# Autodesk Inventor assembly: Z-Axis Assembly
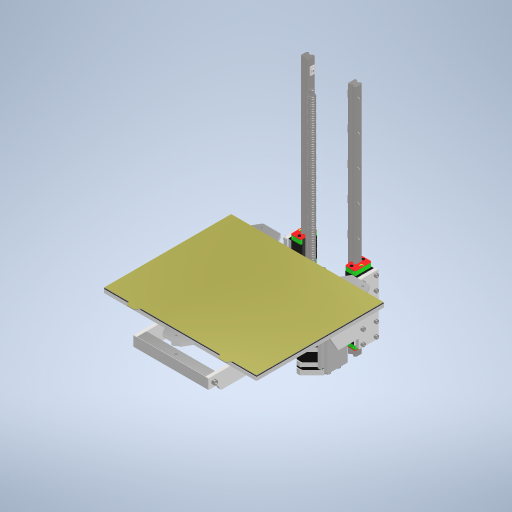
[picture p0: Inventor's stored thumbnail of the model, 512x512]
Saved by Autodesk Inventor 2024 (Build 280153000, 153)
## iProperties
Created: 2024-08-01
Part Number: Z-Axis Assembly
Document SubType Name: Assembly
Designer: Ishaan
Author: Ishaan
## Documents named in this file (32)
- E:\Projects\Axiom--IDEX-3D-Printer\CAD\03 - Z-Axis\Z-Axis Assembly.iam
- E:\Projects\Axiom--IDEX-3D-Printer\CAD\03 - Z-Axis\Z-Axis Motor Plate.ipt
- E:\Projects\Axiom--IDEX-3D-Printer\CAD\00 - COTS Components\FK10\FK10-C5\FK10-C5\FK10-C5.iam
- E:\Projects\Axiom--IDEX-3D-Printer\CAD\00 - COTS Components\5x8 Shaft Coupler\Flexible Coupling 5mm x 8mm.ipt
- E:\Projects\Axiom--IDEX-3D-Printer\CAD\00 - COTS Components\FK10\FK10-C5\Гайка М10х1\Гайка М10х1.iam
- E:\Projects\Axiom--IDEX-3D-Printer\CAD\00 - COTS Components\SFU1204 Ballscrew\1204 Ballscrew.ipt
- E:\Projects\Axiom--IDEX-3D-Printer\CAD\00 - COTS Components\NEMA 17 - Z-Axis Long\NEMA 17 Z-axis Long.ipt
- E:\Projects\Axiom--IDEX-3D-Printer\CAD\03 - Z-Axis\Z-Axis Motor Spacer.ipt
- E:\Projects\Axiom--IDEX-3D-Printer\CAD\00 - COTS Components\NEMA 17 - Z-Axis Short\NEMA 17 Z-axis Short.ipt
- E:\Projects\Axiom--IDEX-3D-Printer\CAD\00 - COTS Components\HGR15 Z-Axis Rail\HGR15-R-700mm\HGR15-R-700mm.iam
- E:\Projects\Axiom--IDEX-3D-Printer\CAD\03 - Z-Axis\Bed Heater.ipt
- E:\Projects\Axiom--IDEX-3D-Printer\CAD\03 - Z-Axis\Bed Magnet.ipt
- E:\Projects\Axiom--IDEX-3D-Printer\CAD\03 - Z-Axis\PEI Bed Surface.ipt
- E:\Projects\Axiom--IDEX-3D-Printer\CAD\03 - Z-Axis\Print Bed.ipt
- E:\Projects\Axiom--IDEX-3D-Printer\CAD\00 - COTS Components\HGH15CA Carriage Block\HGH15CA Hiwin Linear block by proma\HGH15CA Hiwin Linear block by proma.ipt
- E:\Projects\Axiom--IDEX-3D-Printer\CAD\03 - Z-Axis\Z-Axis Bed Plates.ipt
- E:\Projects\Axiom--IDEX-3D-Printer\CAD\00 - COTS Components\2020 Bed Front Extrusion\HFSC5-2020-138.ipt
- E:\Projects\Axiom--IDEX-3D-Printer\CAD\00 - COTS Components\2040 Bed Rear Extrusion\HFSF5-2040-138.ipt
- E:\Projects\Axiom--IDEX-3D-Printer\CAD\00 - COTS Components\1204 Ballscrew Nut\Ballscrew nut 1204 by proma\Ballscrew nut 1204 by proma.ipt
- E:\Projects\Axiom--IDEX-3D-Printer\CAD\03 - Z-Axis\Print Bed Washers.ipt
- E:\Projects\Axiom--IDEX-3D-Printer\CAD\03 - Z-Axis\Z-Axis Nut and Bed Plate RevII.ipt
- E:\Projects\Axiom--IDEX-3D-Printer\CAD\00 - COTS Components\Hardware\M4 T SLOT NUT.ipt
- E:\Projects\Axiom--IDEX-3D-Printer\CAD\00 - COTS Components\Hardware\SHCSM4x14.ipt
- E:\Projects\Axiom--IDEX-3D-Printer\CAD\00 - COTS Components\Hardware\SHCSM5x16.ipt
- E:\Projects\Axiom--IDEX-3D-Printer\CAD\00 - COTS Components\Hardware\SHCSM5x12.ipt
- E:\Projects\Axiom--IDEX-3D-Printer\CAD\00 - COTS Components\Hardware\SHCSM4x10.ipt
- E:\Projects\Axiom--IDEX-3D-Printer\CAD\00 - COTS Components\Hardware\M4 LOCKNUT.ipt
- E:\Projects\Axiom--IDEX-3D-Printer\CAD\00 - COTS Components\Hardware\SHCSM3x8.ipt
- E:\Projects\Axiom--IDEX-3D-Printer\CAD\00 - COTS Components\Hardware\Low Profile M5x12.ipt
- E:\Projects\Axiom--IDEX-3D-Printer\CAD\00 - COTS Components\2040 Z-motor Supports\HFSF5-2040-85.ipt
- E:\Projects\Axiom--IDEX-3D-Printer\CAD\02 - Frame\Printer Base Plate RevII.ipt
- E:\Projects\Axiom--IDEX-3D-Printer\CAD\00 - COTS Components\4080 Z-rail Extrusion\HFSP5-4080-475.ipt
## Components (123 placed, 31 different names)
1. Z-Axis Motor Plate:1 — Insert:1, Insert:2, Insert:7, Insert:8, Insert:74, Insert:75, Insert:76, Insert:77, Insert:86, Insert:87, Insert:88, Insert:89
2. FK10-C5:1 [sub-assembly] — Insert:1, Insert:2, Insert:3, Insert:5, Insert:78, Insert:79, Insert:80, Insert:81
3. Flexible Coupling 5mm x 8mm:1 — Insert:6
4. Гайка М10х1:1 [sub-assembly] — Insert:3
5. 1204 Ballscrew:1 — Insert:5, Insert:6, Z POSITION
6. NEMA 17 Z-axis Long:1 — Insert:9, Insert:10
7. Z-Axis Motor Spacer:1 — Insert:7, Insert:8, Insert:9, Insert:10, Insert:11, Insert:12, Insert:82, Angle:4, Insert:83, Angle:5, Insert:84, Angle:6, Insert:85, Angle:7, Insert:106, Insert:107, Insert:108, Insert:109
8. NEMA 17 Z-axis Short:1 — Insert:11, Insert:12
9. HFSF5-2040-85:1 — Insert:17
10. HFSF5-2040-85:2 — Insert:18
11. Printer Base Plate RevII:1 — Insert:17, Insert:18
12. HFSP5-4080-475:1
13. HGR15-R-700mm:1 [sub-assembly] — Flush:2, Flush:3, Mate:16, Mate:17, Mate:18, Mate:19
14. HGR15-R-700mm:2 [sub-assembly] — Flush:2, Flush:3, Mate:12, Mate:13, Mate:14, Mate:15, Insert:53
15. Bed Heater:1 — Mate:8, Flush:6, Flush:7
16. Bed Magnet:1 — Mate:4, Flush:4, Mate:5, Mate:6
17. PEI Bed Surface:1 — Mate:6, Flush:5, Flush:8, Flush:9
18. Print Bed:1 — Mate:4, Flush:4, Mate:5, Flush:5, Mate:8, Flush:6, Flush:7, Flush:8, Mate:20, Insert:49, Insert:50, Insert:51, Mate:23, Mate:24
19. HGH15CA Hiwin Linear block by proma:1 — Mate:16, Mate:17, Insert:33, Insert:34, Insert:35, Insert:36
20. HGH15CA Hiwin Linear block by proma:2 — Mate:14, Mate:15, Insert:21, Insert:22, Insert:23, Insert:24
21. HGH15CA Hiwin Linear block by proma:3 — Mate:18, Mate:19, Insert:29, Insert:30, Insert:31, Insert:32
22. HGH15CA Hiwin Linear block by proma:4 — Mate:12, Mate:13, Insert:25, Insert:26, Insert:27, Insert:28
23. Z-Axis Bed Plates:1 — Insert:21, Insert:22, Insert:23, Insert:24, Insert:25, Insert:26, Insert:27, Insert:28, Insert:37, Angle:1, Flush:9, Insert:39, Insert:40, Insert:60, Insert:61, Insert:62, Insert:90, Insert:91, Insert:92, Insert:93, Insert:94, Insert:95, Insert:96, Insert:97
24. Z-Axis Bed Plates:2 — Insert:29, Insert:30, Insert:31, Insert:32, Insert:33, Insert:34, Insert:35, Insert:36, Insert:38, Insert:41, Insert:42, Insert:63, Insert:64, Insert:65, Insert:98, Insert:99, Insert:100, Insert:101, Insert:102, Insert:103, Insert:104, Insert:105
25. HFSC5-2020-138:1 — Insert:37, Insert:38, Angle:1, Mate:20
26. HFSF5-2040-138:1 — Insert:39, Insert:40, Insert:41, Insert:42
27. Z-Axis Nut and Bed Plate RevII:1 — Mate:23, Mate:24, Insert:66, Insert:67, Insert:68, Insert:69, Insert:70, Insert:71, Insert:72, Insert:73
28. Ballscrew nut 1204 by proma:1 — Z POSITION, Insert:54, Insert:55, Insert:56, Insert:57, Insert:58, Insert:59
29. Print Bed Washers:1 — Insert:49
30. Print Bed Washers:2 — Insert:50
31. Print Bed Washers:3 — Insert:51
32. SHCSM4x10:13 — Insert:103
33. SHCSM4x10:14 — Insert:102
34. SHCSM4x10:15 — Insert:100
35. SHCSM4x10:16 — Insert:99
36. SHCSM4x10:17 — Insert:98
37. SHCSM4x10:18 — Insert:101
38. SHCSM4x10:19 — Insert:104
39. SHCSM4x10:20 — Insert:105
40. SHCSM3x8:1 — Insert:106
41. SHCSM3x8:2 — Insert:107
42. SHCSM3x8:3 — Insert:109
43. SHCSM3x8:4 — Insert:108
44. Low Profile M5x12:1
45. Low Profile M5x12:2
46. Low Profile M5x12:3
47. Low Profile M5x12:4
48. SHCSM5x12:1 — Insert:66
49. SHCSM5x12:2 — Insert:67
50. SHCSM5x12:3 — Insert:73
51. SHCSM5x12:4 — Insert:69
52. SHCSM5x12:5 — Insert:68
53. SHCSM5x12:6 — Insert:70
54. SHCSM5x12:7 — Insert:72
55. SHCSM5x12:8 — Insert:71
56. SHCSM5x16:7 — Insert:74
57. SHCSM5x16:8 — Insert:75
58. SHCSM5x16:9 — Insert:76
59. SHCSM5x16:10 — Insert:77
60. SHCSM4x10:1 — Insert:78
61. SHCSM4x10:2 — Insert:79
62. SHCSM4x10:3 — Insert:80
63. SHCSM4x10:4 — Insert:81
64. M4 LOCKNUT:1 — Insert:82, Angle:4
65. M4 LOCKNUT:2 — Insert:83, Angle:5
66. M4 LOCKNUT:3 — Insert:84, Angle:6
67. M4 LOCKNUT:4 — Insert:85, Angle:7
68. SHCSM4x14:23 — Insert:86
69. SHCSM4x14:24 — Insert:87
70. SHCSM4x14:25 — Insert:88
71. SHCSM4x14:26 — Insert:89
72. SHCSM4x10:5 — Insert:94
73. SHCSM4x10:6 — Insert:95
74. SHCSM4x10:7 — Insert:96
75. SHCSM4x10:8 — Insert:97
76. SHCSM4x10:9 — Insert:93
77. SHCSM4x10:10 — Insert:92
78. SHCSM4x10:11 — Insert:91
79. SHCSM4x10:12 — Insert:90
80. SHCSM5x16:1 — Insert:60
81. SHCSM5x16:2 — Insert:61
82. SHCSM5x16:3 — Insert:62
83. SHCSM5x16:4 — Insert:63
84. SHCSM5x16:5 — Insert:65
85. SHCSM5x16:6 — Insert:64
86. SHCSM4x14:17 — Insert:56
87. SHCSM4x14:18 — Insert:57
88. SHCSM4x14:19 — Insert:55
89. SHCSM4x14:20 — Insert:58
90. SHCSM4x14:21 — Insert:54
91. SHCSM4x14:22 — Insert:59
92. SHCSM4x14:1 — Insert:53, Mate:27
93. M4 T SLOT NUT:9 — Mate:27
94. M4 T SLOT NUT:1 — Mate:25
95. SHCSM4x14:2 — Mate:25
96. SHCSM4x14:3
97. M4 T SLOT NUT:10
98. M4 T SLOT NUT:11
99. SHCSM4x14:4
100. SHCSM4x14:5
101. M4 T SLOT NUT:12
102. M4 T SLOT NUT:13
103. SHCSM4x14:6
104. SHCSM4x14:7
105. M4 T SLOT NUT:14
106. M4 T SLOT NUT:15
107. SHCSM4x14:8
108. SHCSM4x14:9
109. M4 T SLOT NUT:16
110. M4 T SLOT NUT:17
111. SHCSM4x14:10
112. SHCSM4x14:11
113. M4 T SLOT NUT:18
114. M4 T SLOT NUT:19
115. SHCSM4x14:12
116. SHCSM4x14:13
117. M4 T SLOT NUT:20
118. M4 T SLOT NUT:21
119. SHCSM4x14:14
120. SHCSM4x14:15
121. M4 T SLOT NUT:22
122. M4 T SLOT NUT:23
123. SHCSM4x14:16
## Component patterns: (8 elements, first: SHCSM4x14:1 + M4 T SLOT NUT:9 + M4 T SLOT NUT:1 + SHCSM4x14:2)
## Relationships (154: Insert 112, Mate 23, Flush 12, Angle 7)
- Insert:1: Z-Axis Motor Plate:1 ↔ FK10-C5:1
- Insert:2: Z-Axis Motor Plate:1 ↔ FK10-C5:1
- Insert:3: FK10-C5:1 ↔ Гайка М10х1:1
- Insert:5: FK10-C5:1 ↔ 1204 Ballscrew:1
- Insert:6 (1 mm): Flexible Coupling 5mm x 8mm:1 ↔ 1204 Ballscrew:1
- Insert:7: Z-Axis Motor Plate:1 ↔ Z-Axis Motor Spacer:1
- Insert:8: Z-Axis Motor Plate:1 ↔ Z-Axis Motor Spacer:1
- Insert:9: NEMA 17 Z-axis Long:1 ↔ Z-Axis Motor Spacer:1
- Insert:10: NEMA 17 Z-axis Long:1 ↔ Z-Axis Motor Spacer:1
- Insert:11: Z-Axis Motor Spacer:1 ↔ NEMA 17 Z-axis Short:1
- Insert:12: Z-Axis Motor Spacer:1 ↔ NEMA 17 Z-axis Short:1
- [Insert]: Z-Axis Motor Plate:1 ↔ HFSF5-2040-85:2
- [Insert]: Z-Axis Motor Plate:1 ↔ HFSF5-2040-85:2
- [Insert]: Z-Axis Motor Plate:1 ↔ HFSF5-2040-85:1
- [Insert]: Z-Axis Motor Plate:1 ↔ HFSF5-2040-85:1
- Insert:17: HFSF5-2040-85:1 ↔ Printer Base Plate RevII:1
- Insert:18: HFSF5-2040-85:2 ↔ Printer Base Plate RevII:1
- [Insert]: Printer Base Plate RevII:1 ↔ HFSP5-4080-475:1
- [Insert]: Printer Base Plate RevII:1 ↔ HFSP5-4080-475:1
- [Mate]: HFSP5-4080-475:1 ↔ HGR15-R-700mm:2
- [Mate]: HFSP5-4080-475:1 ↔ HGR15-R-700mm:1
- [Flush] (2.5 mm): HFSP5-4080-475:1 ↔ HGR15-R-700mm:1
- Flush:2: HGR15-R-700mm:1 ↔ HGR15-R-700mm:2
- Flush:3: HGR15-R-700mm:1 ↔ HGR15-R-700mm:2
- Mate:4: Bed Magnet:1 ↔ Print Bed:1
- Flush:4: Bed Magnet:1 ↔ Print Bed:1
- Mate:5: Bed Magnet:1 ↔ Print Bed:1
- Mate:6: Bed Magnet:1 ↔ PEI Bed Surface:1
- Flush:5: PEI Bed Surface:1 ↔ Print Bed:1
- Mate:8: Bed Heater:1 ↔ Print Bed:1
- Flush:6: Bed Heater:1 ↔ Print Bed:1
- Flush:7: Bed Heater:1 ↔ Print Bed:1
- Flush:8: PEI Bed Surface:1 ↔ Print Bed:1
- Mate:12: HGR15-R-700mm:2 ↔ HGH15CA Hiwin Linear block by proma:4
- Mate:13: HGR15-R-700mm:2 ↔ HGH15CA Hiwin Linear block by proma:4
- Mate:14: HGR15-R-700mm:2 ↔ HGH15CA Hiwin Linear block by proma:2
- Mate:15: HGR15-R-700mm:2 ↔ HGH15CA Hiwin Linear block by proma:2
- Mate:16: HGR15-R-700mm:1 ↔ HGH15CA Hiwin Linear block by proma:1
- Mate:17: HGR15-R-700mm:1 ↔ HGH15CA Hiwin Linear block by proma:1
- Mate:18: HGR15-R-700mm:1 ↔ HGH15CA Hiwin Linear block by proma:3
- Mate:19: HGR15-R-700mm:1 ↔ HGH15CA Hiwin Linear block by proma:3
- Insert:21: HGH15CA Hiwin Linear block by proma:2 ↔ Z-Axis Bed Plates:1
- Insert:22: HGH15CA Hiwin Linear block by proma:2 ↔ Z-Axis Bed Plates:1
- Insert:23: HGH15CA Hiwin Linear block by proma:2 ↔ Z-Axis Bed Plates:1
- Insert:24: HGH15CA Hiwin Linear block by proma:2 ↔ Z-Axis Bed Plates:1
- Insert:25: HGH15CA Hiwin Linear block by proma:4 ↔ Z-Axis Bed Plates:1
- Insert:26: HGH15CA Hiwin Linear block by proma:4 ↔ Z-Axis Bed Plates:1
- Insert:27: HGH15CA Hiwin Linear block by proma:4 ↔ Z-Axis Bed Plates:1
- Insert:28: HGH15CA Hiwin Linear block by proma:4 ↔ Z-Axis Bed Plates:1
- Insert:29: HGH15CA Hiwin Linear block by proma:3 ↔ Z-Axis Bed Plates:2
- Insert:30: HGH15CA Hiwin Linear block by proma:3 ↔ Z-Axis Bed Plates:2
- Insert:31: HGH15CA Hiwin Linear block by proma:3 ↔ Z-Axis Bed Plates:2
- Insert:32: HGH15CA Hiwin Linear block by proma:3 ↔ Z-Axis Bed Plates:2
- Insert:33: HGH15CA Hiwin Linear block by proma:1 ↔ Z-Axis Bed Plates:2
- Insert:34: HGH15CA Hiwin Linear block by proma:1 ↔ Z-Axis Bed Plates:2
- Insert:35: HGH15CA Hiwin Linear block by proma:1 ↔ Z-Axis Bed Plates:2
- Insert:36: HGH15CA Hiwin Linear block by proma:1 ↔ Z-Axis Bed Plates:2
- Insert:37: Z-Axis Bed Plates:1 ↔ HFSC5-2020-138:1
- Insert:38: Z-Axis Bed Plates:2 ↔ HFSC5-2020-138:1
- Angle:1 (0 deg): Z-Axis Bed Plates:1 ↔ HFSC5-2020-138:1
- Mate:20: Print Bed:1 ↔ HFSC5-2020-138:1
- Flush:9: PEI Bed Surface:1 ↔ Z-Axis Bed Plates:1
- Insert:39: Z-Axis Bed Plates:1 ↔ HFSF5-2040-138:1
- Insert:40: Z-Axis Bed Plates:1 ↔ HFSF5-2040-138:1
- Insert:41: Z-Axis Bed Plates:2 ↔ HFSF5-2040-138:1
- Insert:42: Z-Axis Bed Plates:2 ↔ HFSF5-2040-138:1
- [Mate]: HFSF5-2040-138:1 ↔ Z-Axis Nut and Bed Plate RevII:1
- [Flush]: HFSF5-2040-138:1 ↔ Z-Axis Nut and Bed Plate RevII:1
- [Mate]: HFSF5-2040-138:1 ↔ Z-Axis Nut and Bed Plate RevII:1
- [Insert]: Z-Axis Nut and Bed Plate RevII:1 ↔ Ballscrew nut 1204 by proma:1
- [Insert]: Z-Axis Nut and Bed Plate RevII:1 ↔ Ballscrew nut 1204 by proma:1
- [Insert]: Z-Axis Nut and Bed Plate RevII:1 ↔ Ballscrew nut 1204 by proma:1
- [Insert]: Z-Axis Nut and Bed Plate RevII:1 ↔ Ballscrew nut 1204 by proma:1
- [Insert]: Z-Axis Nut and Bed Plate RevII:1 ↔ Ballscrew nut 1204 by proma:1
- [Insert]: Z-Axis Nut and Bed Plate RevII:1 ↔ Ballscrew nut 1204 by proma:1
- Z POSITION [Flush]: 1204 Ballscrew:1 ↔ Ballscrew nut 1204 by proma:1
- [Flush] (10 mm): HFSP5-4080-475:1 ↔ HGR15-R-700mm:2
- Insert:49: Print Bed:1 ↔ Print Bed Washers:1
- Insert:50: Print Bed:1 ↔ Print Bed Washers:2
- Insert:51: Print Bed:1 ↔ Print Bed Washers:3
- Mate:23: Print Bed:1 ↔ Z-Axis Nut and Bed Plate RevII:1
- Mate:24: Print Bed:1 ↔ Z-Axis Nut and Bed Plate RevII:1
- [Insert]: HGR15-R-700mm:1 ↔ SHCSM4x14:2
- Mate:25: M4 T SLOT NUT:1 ↔ SHCSM4x14:2
- [Mate]: HFSP5-4080-475:1 ↔ M4 T SLOT NUT:1
- [Angle] (0 deg): HFSP5-4080-475:1 ↔ M4 T SLOT NUT:1
- Insert:53: HGR15-R-700mm:2 ↔ SHCSM4x14:1
- Mate:27: SHCSM4x14:1 ↔ M4 T SLOT NUT:9
- [Mate]: HFSP5-4080-475:1 ↔ M4 T SLOT NUT:9
- [Angle] (0 deg): HFSP5-4080-475:1 ↔ M4 T SLOT NUT:9
- Insert:54: Ballscrew nut 1204 by proma:1 ↔ SHCSM4x14:21
- Insert:55: Ballscrew nut 1204 by proma:1 ↔ SHCSM4x14:19
- Insert:56: Ballscrew nut 1204 by proma:1 ↔ SHCSM4x14:17
- Insert:57: Ballscrew nut 1204 by proma:1 ↔ SHCSM4x14:18
- Insert:58: Ballscrew nut 1204 by proma:1 ↔ SHCSM4x14:20
- Insert:59: Ballscrew nut 1204 by proma:1 ↔ SHCSM4x14:22
- Insert:60: Z-Axis Bed Plates:1 ↔ SHCSM5x16:1
- Insert:61: Z-Axis Bed Plates:1 ↔ SHCSM5x16:2
- Insert:62: Z-Axis Bed Plates:1 ↔ SHCSM5x16:3
- Insert:63: Z-Axis Bed Plates:2 ↔ SHCSM5x16:4
- Insert:64: Z-Axis Bed Plates:2 ↔ SHCSM5x16:6
- Insert:65: Z-Axis Bed Plates:2 ↔ SHCSM5x16:5
- Insert:66: Z-Axis Nut and Bed Plate RevII:1 ↔ SHCSM5x12:1
- Insert:67: Z-Axis Nut and Bed Plate RevII:1 ↔ SHCSM5x12:2
- Insert:68: Z-Axis Nut and Bed Plate RevII:1 ↔ SHCSM5x12:5
- Insert:69: Z-Axis Nut and Bed Plate RevII:1 ↔ SHCSM5x12:4
- Insert:70: Z-Axis Nut and Bed Plate RevII:1 ↔ SHCSM5x12:6
- Insert:71: Z-Axis Nut and Bed Plate RevII:1 ↔ SHCSM5x12:8
- Insert:72: Z-Axis Nut and Bed Plate RevII:1 ↔ SHCSM5x12:7
- Insert:73: Z-Axis Nut and Bed Plate RevII:1 ↔ SHCSM5x12:3
- Insert:74: Z-Axis Motor Plate:1 ↔ SHCSM5x16:7
- Insert:75: Z-Axis Motor Plate:1 ↔ SHCSM5x16:8
- Insert:76: Z-Axis Motor Plate:1 ↔ SHCSM5x16:9
- Insert:77: Z-Axis Motor Plate:1 ↔ SHCSM5x16:10
- Insert:78: FK10-C5:1 ↔ SHCSM4x10:1
- Insert:79: FK10-C5:1 ↔ SHCSM4x10:2
- Insert:80: FK10-C5:1 ↔ SHCSM4x10:3
- Insert:81: FK10-C5:1 ↔ SHCSM4x10:4
- Insert:82: Z-Axis Motor Spacer:1 ↔ M4 LOCKNUT:1
- Angle:4 (0 deg): Z-Axis Motor Spacer:1 ↔ M4 LOCKNUT:1
- Insert:83: Z-Axis Motor Spacer:1 ↔ M4 LOCKNUT:2
- Angle:5 (0 deg): Z-Axis Motor Spacer:1 ↔ M4 LOCKNUT:2
- Insert:84: Z-Axis Motor Spacer:1 ↔ M4 LOCKNUT:3
- Angle:6 (0 deg): Z-Axis Motor Spacer:1 ↔ M4 LOCKNUT:3
- Insert:85: Z-Axis Motor Spacer:1 ↔ M4 LOCKNUT:4
- Angle:7 (0 deg): Z-Axis Motor Spacer:1 ↔ M4 LOCKNUT:4
- Insert:86: Z-Axis Motor Plate:1 ↔ SHCSM4x14:23
- Insert:87: Z-Axis Motor Plate:1 ↔ SHCSM4x14:24
- Insert:88: Z-Axis Motor Plate:1 ↔ SHCSM4x14:25
- Insert:89: Z-Axis Motor Plate:1 ↔ SHCSM4x14:26
- Insert:90: Z-Axis Bed Plates:1 ↔ SHCSM4x10:12
- Insert:91: Z-Axis Bed Plates:1 ↔ SHCSM4x10:11
- Insert:92: Z-Axis Bed Plates:1 ↔ SHCSM4x10:10
- Insert:93: Z-Axis Bed Plates:1 ↔ SHCSM4x10:9
- Insert:94: Z-Axis Bed Plates:1 ↔ SHCSM4x10:5
- Insert:95: Z-Axis Bed Plates:1 ↔ SHCSM4x10:6
- Insert:96: Z-Axis Bed Plates:1 ↔ SHCSM4x10:7
- Insert:97: Z-Axis Bed Plates:1 ↔ SHCSM4x10:8
- Insert:98: Z-Axis Bed Plates:2 ↔ SHCSM4x10:17
- Insert:99: Z-Axis Bed Plates:2 ↔ SHCSM4x10:16
- Insert:100: Z-Axis Bed Plates:2 ↔ SHCSM4x10:15
- Insert:101: Z-Axis Bed Plates:2 ↔ SHCSM4x10:18
- Insert:102: Z-Axis Bed Plates:2 ↔ SHCSM4x10:14
- Insert:103: Z-Axis Bed Plates:2 ↔ SHCSM4x10:13
- Insert:104: Z-Axis Bed Plates:2 ↔ SHCSM4x10:19
- Insert:105: Z-Axis Bed Plates:2 ↔ SHCSM4x10:20
- Insert:106: Z-Axis Motor Spacer:1 ↔ SHCSM3x8:1
- Insert:107: Z-Axis Motor Spacer:1 ↔ SHCSM3x8:2
- Insert:108: Z-Axis Motor Spacer:1 ↔ SHCSM3x8:4
- Insert:109: Z-Axis Motor Spacer:1 ↔ SHCSM3x8:3
- [Insert] (6.35 mm): HFSF5-2040-85:1 ↔ Low Profile M5x12:1
- [Insert] (6.35 mm): HFSF5-2040-85:1 ↔ Low Profile M5x12:2
- [Insert] (6.35 mm): HFSF5-2040-85:2 ↔ Low Profile M5x12:3
- [Insert] (6.35 mm): HFSF5-2040-85:2 ↔ Low Profile M5x12:4
